# Autodesk Inventor assembly: final assembly
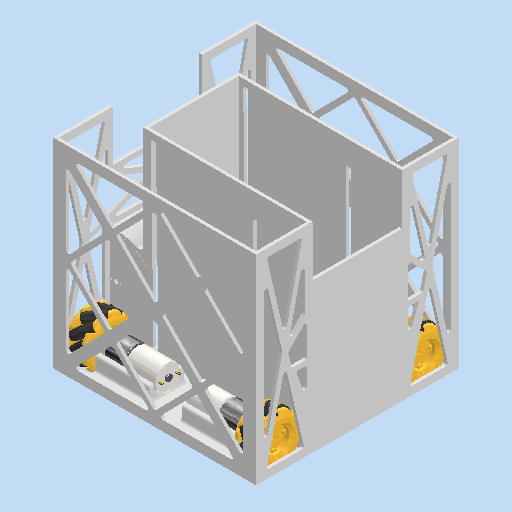
[picture p0: Inventor's stored thumbnail of the model, 512x512]
Saved by Autodesk Inventor 2026 (Build 300175000, 175)
## iProperties
Created: 2026-02-10
Part Number: final assembly
Document SubType Name: Assembly
Designer: mones
Author: mones
## Documents named in this file (14)
- C:\Users\mones\OneDrive - Northeastern University\unibots\Unibots_NULondon\hardware\final assembly\final assembly.iam
- C:\Users\mones\OneDrive - Northeastern University\unibots\Unibots_NULondon\hardware\chassis\final\inside walls left.ipt
- inside walls left.ipt
- C:\Users\mones\OneDrive - Northeastern University\unibots\Unibots_NULondon\hardware\chassis\final\inside walls right.ipt
- C:\Users\mones\OneDrive - Northeastern University\unibots\Unibots_NULondon\hardware\motor_mounts\bottom plate left\bottom plate.ipt
- C:\Users\mones\OneDrive - Northeastern University\unibots\Unibots_NULondon\hardware\chassis\final\back plate.ipt
- C:\Users\mones\OneDrive - Northeastern University\unibots\Unibots_NULondon\hardware\chassis\final\front plate.ipt
- C:\Users\mones\OneDrive - Northeastern University\unibots\Unibots_NULondon\hardware\chassis\final\left plate.ipt
- C:\Users\mones\OneDrive - Northeastern University\unibots\Unibots_NULondon\hardware\motor_mounts\25ga-370-280-rpm-dc-motor-1.snapshot.1\25ga-370-280-rpm-dc Motor.ipt
- C:\Users\mones\OneDrive - Northeastern University\unibots\Unibots_NULondon\hardware\chassis\Mecanum Left v5\Mecanum Left.iam
- C:\Users\mones\OneDrive - Northeastern University\unibots\Unibots_NULondon\hardware\chassis\Mecanum Left v5\Mecanum Left_MIR.iam
- C:\Users\mones\OneDrive - Northeastern University\unibots\Unibots_NULondon\hardware\chassis\lift plate.ipt
- C:\Users\mones\OneDrive - Northeastern University\unibots\Unibots_NULondon\hardware\chassis\final\bridge plate.ipt
- C:\Users\mones\OneDrive - Northeastern University\unibots\Unibots_NULondon\hardware\chassis\final\right plate.ipt
## Components (18 placed, 12 different names)
1. inside walls left:1 — Mate:1, Mate:2, Mate:8, Mate:9, Mate:10
2. inside walls:1 — Mate:3, Mate:4, Mate:5, Mate:6, Mate:7, Insert:5, Insert:6, Flush:1, Flush:2, Flush:3
3. bottom plate:1 — Mate:3, Mate:4, Mate:21, Mate:22, Mate:23, Mate:24, Mate:25, Mate:26, Insert:1, Insert:4
4. bottom plate:2 — Mate:1, Mate:2, Mate:15, Mate:16, Mate:17, Mate:18, Mate:19, Mate:20, Insert:2, Insert:3
5. back plate:1 — Mate:5, Mate:6, Mate:7, Mate:8, Flush:4, Flush:5, Flush:6
6. front plate:1 — Mate:9, Mate:10, Mate:11, Mate:12
7. left plate:1 — Mate:11, Mate:12
8. 25ga-370-280-rpm-dc Motor:1 — Mate:15, Mate:16, Mate:17
9. 25ga-370-280-rpm-dc Motor:2 — Mate:18, Mate:19, Mate:20
10. 25ga-370-280-rpm-dc Motor:3 — Mate:21, Mate:22, Mate:23
11. 25ga-370-280-rpm-dc Motor:4 — Mate:24, Mate:25, Mate:26
12. Mecanum Left:1 [sub-assembly] — Insert:2
13. Mecanum Left_MIR:1 [sub-assembly] — Insert:4
14. Mecanum Left:2 [sub-assembly] — Insert:1
15. Mecanum Left_MIR:2 [sub-assembly] — Insert:3
16. lift plate:1 — Insert:5, Insert:6
17. bridge plate:1 — Flush:1, Flush:2, Flush:3
18. right plate:1 — Flush:4, Flush:5, Flush:6
## Relationships (36: Mate 24, Insert 6, Flush 6)
- Mate:1: inside walls left:1 ↔ bottom plate:2
- Mate:2: inside walls left:1 ↔ bottom plate:2
- Mate:3: inside walls:1 ↔ bottom plate:1
- Mate:4: inside walls:1 ↔ bottom plate:1
- Mate:5: inside walls:1 ↔ back plate:1
- Mate:6: inside walls:1 ↔ back plate:1
- Mate:7: inside walls:1 ↔ back plate:1
- Mate:8: inside walls left:1 ↔ back plate:1
- Mate:9: inside walls left:1 ↔ front plate:1
- Mate:10: inside walls left:1 ↔ front plate:1
- Mate:11: front plate:1 ↔ left plate:1
- Mate:12: front plate:1 ↔ left plate:1
- Mate:15: bottom plate:2 ↔ 25ga-370-280-rpm-dc Motor:1
- Mate:16: bottom plate:2 ↔ 25ga-370-280-rpm-dc Motor:1
- Mate:17: bottom plate:2 ↔ 25ga-370-280-rpm-dc Motor:1
- Mate:18: bottom plate:2 ↔ 25ga-370-280-rpm-dc Motor:2
- Mate:19: bottom plate:2 ↔ 25ga-370-280-rpm-dc Motor:2
- Mate:20: bottom plate:2 ↔ 25ga-370-280-rpm-dc Motor:2
- Mate:21: bottom plate:1 ↔ 25ga-370-280-rpm-dc Motor:3
- Mate:22: bottom plate:1 ↔ 25ga-370-280-rpm-dc Motor:3
- Mate:23: bottom plate:1 ↔ 25ga-370-280-rpm-dc Motor:3
- Mate:24: bottom plate:1 ↔ 25ga-370-280-rpm-dc Motor:4
- Mate:25: bottom plate:1 ↔ 25ga-370-280-rpm-dc Motor:4
- Mate:26: bottom plate:1 ↔ 25ga-370-280-rpm-dc Motor:4
- Insert:1 (1 mm): bottom plate:1 ↔ Mecanum Left:2
- Insert:2 (1 mm): bottom plate:2 ↔ Mecanum Left:1
- Insert:3 (1 mm): bottom plate:2 ↔ Mecanum Left_MIR:2
- Insert:4 (1 mm): bottom plate:1 ↔ Mecanum Left_MIR:1
- Insert:5: inside walls:1 ↔ lift plate:1
- Insert:6: inside walls:1 ↔ lift plate:1
- Flush:1: inside walls:1 ↔ bridge plate:1
- Flush:2: inside walls:1 ↔ bridge plate:1
- Flush:3: inside walls:1 ↔ bridge plate:1
- Flush:4: back plate:1 ↔ right plate:1
- Flush:5: back plate:1 ↔ right plate:1
- Flush:6: back plate:1 ↔ right plate:1
